# Autodesk Inventor assembly: E3Dv6_1_75mm_Threaded_Heatsink
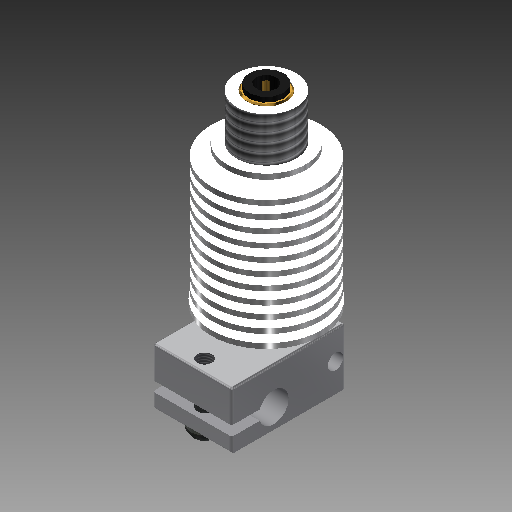
[picture p0: Inventor's stored thumbnail of the model, 512x512]
Saved by Autodesk Inventor 2019 (Build 230136000, 136)
## iProperties
Created: 2018-10-01
Part Number: E3Dv6_1_75mm_Threaded_Heatsink
Document SubType Name: Assembly
Designer: Ax
Author: Ax
## Documents named in this file (8)
- C:\Users\Ax\Google Drive\Inventor\Library\E3Dv6_1_75mm_Threaded_Heatsink .iam
- C:\Users\Ax\Google Drive\Inventor\Library\Collet.ipt
- C:\Users\Ax\Google Drive\Inventor\Library\Threaded Heatsink.ipt
- C:\Users\Ax\Google Drive\Inventor\Library\E3Dv6_heatbreak.ipt
- C:\Users\Ax\Google Drive\Inventor\Library\E3Dv6_Heater_Block.ipt
- C:\Users\Ax\Google Drive\Inventor\Library\E3Dv6_Nozzle.ipt
- C:\Users\Ax\Google Drive\Autodesk\Content Center Files\R2017\en-US\ISO 7380-1\ISO 7380-1 - M3 x 8.ipt
- C:\Users\Ax\Google Drive\Autodesk\Content Center Files\R2017\en-US\DIN EN ISO 4029\DIN EN ISO 4029 - M3  x  4.ipt
## Components (7 placed, 7 different names)
1. Collet:1 — Mate:1, Mate:2
2. Threaded Heatsink:1 — Mate:1, Mate:2, Insert:1
3. E3Dv6_heatbreak:1 — Insert:1, Mate:5, Mate:6
4. E3Dv6_Heater_Block:1 — Mate:3, Mate:4, Mate:6, Insert:2, Insert:3
5. E3Dv6_Nozzle:1 — Mate:3, Mate:4, Mate:5
6. ISO 7380-1 M3 x 8:1 — Insert:2
7. DIN EN ISO 4029 M3  x  4:1 — Insert:3
## Relationships (9: Mate 6, Insert 3)
- Mate:1: Collet:1 ↔ Threaded Heatsink:1
- Mate:2: Collet:1 ↔ Threaded Heatsink:1
- Insert:1: Threaded Heatsink:1 ↔ E3Dv6_heatbreak:1
- Mate:3: E3Dv6_Heater_Block:1 ↔ E3Dv6_Nozzle:1
- Mate:4: E3Dv6_Heater_Block:1 ↔ E3Dv6_Nozzle:1
- Mate:5: E3Dv6_heatbreak:1 ↔ E3Dv6_Nozzle:1
- Mate:6: E3Dv6_heatbreak:1 ↔ E3Dv6_Heater_Block:1
- Insert:2: E3Dv6_Heater_Block:1 ↔ ISO 7380-1 M3 x 8:1
- Insert:3: E3Dv6_Heater_Block:1 ↔ DIN EN ISO 4029 M3  x  4:1
